# Autodesk Inventor assembly: AMT103Encoder
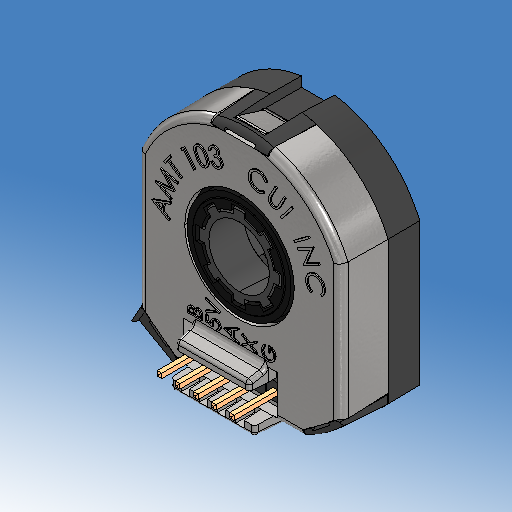
[picture p0: Inventor's stored thumbnail of the model, 512x512]
Saved by Autodesk Inventor 2025 (Build 290162000, 162)
## iProperties
Created: 2024-06-19
Part Number: AMT103Encoder
Document SubType Name: Assembly
Designer: seene
Author: seene
## Documents named in this file (3)
- C:\Users\seene\Desktop\Stony Brook\SBRT\RCR_Dexter\AMT103Encoder.iam
- C:\Users\seene\Desktop\Stony Brook\SBRT\RCR_Dexter\Drive\v1\amt103-v_25 MODIFIED FOR TETRIX(2).ipt
- C:\Users\seene\Desktop\Stony Brook\SBRT\RCR_Dexter\Drive\v1\amt103-v unit only.ipt
## Components (2 placed, 2 different names)
1. amt103-v_25 MODIFIED FOR TETRIX(2):1 — Mate:1, Mate:2
2. amt103-v unit only:1 — Mate:1, Mate:2
## Relationships (2: Mate 2)
- Mate:1: amt103-v_25 MODIFIED FOR TETRIX(2):1 ↔ amt103-v unit only:1
- Mate:2: amt103-v_25 MODIFIED FOR TETRIX(2):1 ↔ amt103-v unit only:1
